# Autodesk Inventor assembly: counter_sensors_assembly
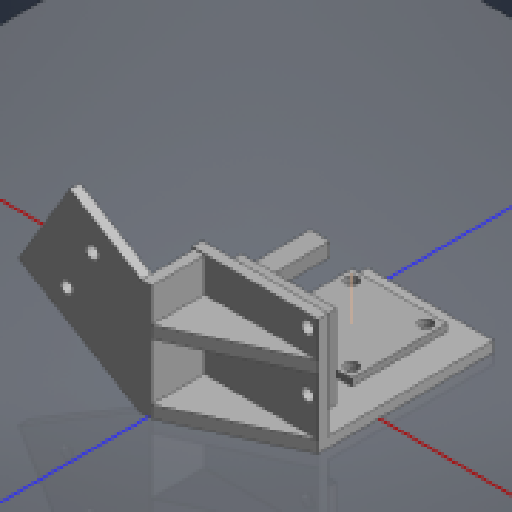
[picture p0: Inventor's stored thumbnail of the model, 512x512]
Saved by Autodesk Inventor 2024 (Build 280153000, 153)
## iProperties
Created: 2026-03-30
Part Number: counter_sensors_assembly
Document SubType Name: Assembly
Designer: schar
Author: schar
## Documents named in this file (4)
- C:\Users\schar\Desktop\FloatingFace\models\counter_sensors_assembly.iam
- C:\Users\schar\Desktop\FloatingFace\models\counter_sensor_holders.ipt
- C:\Users\schar\Desktop\FloatingFace\models\magentic_encoder_modell.ipt
- C:\Users\schar\Desktop\FloatingFace\models\lichtschrankenmodulmodell.ipt
## Components (3 placed, 3 different names)
1. counter_sensor_holders:1 — Mate:1, Mate:2, Mate:3, Mate:4, Mate:5, Mate:6
2. magentic_encoder_modell:1 — Mate:1, Mate:2, Mate:6
3. lichtschrankenmodulmodell:1 — Mate:3, Mate:4, Mate:5
## Relationships (6: Mate 6)
- Mate:1: counter_sensor_holders:1 ↔ magentic_encoder_modell:1
- Mate:2: counter_sensor_holders:1 ↔ magentic_encoder_modell:1
- Mate:3: counter_sensor_holders:1 ↔ lichtschrankenmodulmodell:1
- Mate:4: counter_sensor_holders:1 ↔ lichtschrankenmodulmodell:1
- Mate:5: counter_sensor_holders:1 ↔ lichtschrankenmodulmodell:1
- Mate:6: counter_sensor_holders:1 ↔ magentic_encoder_modell:1
